# Autodesk Inventor assembly: cosel-psu-din-clip
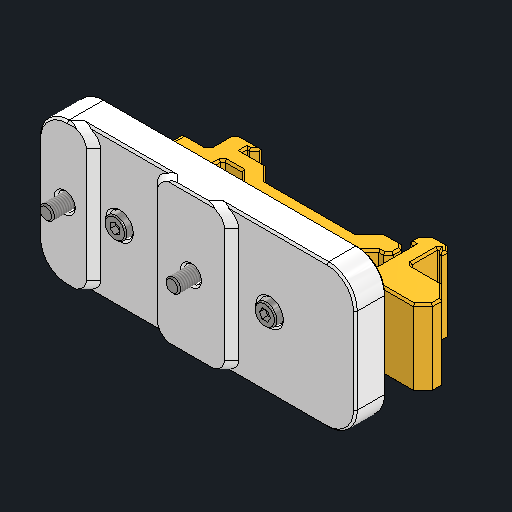
[picture p0: Inventor's stored thumbnail of the model, 512x512]
Saved by Autodesk Inventor 2027.1 (Build 311270010, 270A)
## iProperties
Created: 2026-03-04
Part Number: cosel-psu-din-clip
Document SubType Name: Assembly
Designer: kuzmin
Author: kuzmin
## Documents named in this file (5)
- C:\Users\queezz\Dropbox\Drawings\PIHTI\ElectronicsBox\Win-GPIO-Box\cosel-psu-din-clip.iam
- C:\Users\queezz\Dropbox\Drawings\PIHTI\ElectronicsBox\Win-GPIO-Box\cosel-psu-bracket.ipt
- C:\Users\queezz\Dropbox\Drawings\PIHTI\ContentCenter\Fastners\M2.5x10-SHCS.ipt
- C:\Users\queezz\Dropbox\Drawings\PIHTI\ContentCenter\Fastners\M3x12-SHCS.ipt
- C:\Users\queezz\Dropbox\Drawings\PIHTI\ElectronicsBox\TempController\Wide Din Clip V1.ipt
## Components (6 placed, 4 different names)
1. cosel-psu-bracket:1 — Rigid:2, Rigid:3, Mate:1, Mate:2, Rigid:4, Rigid:5
2. Wide Din Clip V1:1 — Rigid:5
3. BS EN ISO 4762 - Metric M2,5 x 10:1 — Rigid:2
4. BS EN ISO 4762 - Metric M2,5 x 10:2 — Rigid:3
5. AS 1420 - Metric M3 x 12:1 — Mate:1, Mate:2
6. AS 1420 - Metric M3 x 12:2 — Rigid:4
## Relationships (6: WeldJoint 4, Mate 2)
- Rigid:2 [WeldJoint]: cosel-psu-bracket:1 ↔ BS EN ISO 4762 - Metric M2,5 x 10:1
- Rigid:3 [WeldJoint]: cosel-psu-bracket:1 ↔ BS EN ISO 4762 - Metric M2,5 x 10:2
- Mate:1: cosel-psu-bracket:1 ↔ AS 1420 - Metric M3 x 12:1
- Mate:2: cosel-psu-bracket:1 ↔ AS 1420 - Metric M3 x 12:1
- Rigid:4 [WeldJoint]: cosel-psu-bracket:1 ↔ AS 1420 - Metric M3 x 12:2
- Rigid:5 [WeldJoint]: cosel-psu-bracket:1 ↔ Wide Din Clip V1:1
